# Autodesk Inventor assembly: E001-Chambre
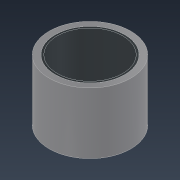
[picture p0: Inventor's stored thumbnail of the model, 180x180]
Saved by Autodesk Inventor 2021.3 (Build 253353000, 353)
## iProperties
Created: 2022-03-31
Part Number: E001-Chambre
Document SubType Name: Assembly
Designer: remi
Author: remi
## Documents named in this file (3)
- C:\Users\remi\OneDrive\Documents\Cours\05-HEVS\S2fb\mechanic\CCo\project\Compressor\E001-Chambre.iam
- C:\Users\remi\OneDrive\Documents\Cours\05-HEVS\S2fb\mechanic\CCo\project\Compressor\P002-Bati_chambre.ipt
- C:\Users\remi\OneDrive\Documents\Cours\05-HEVS\S2fb\mechanic\CCo\project\Compressor\P001-Couverture.ipt
## Components (2 placed, 2 different names)
1. P002-Bati_chambre:1 — Mate:1, Flush:1
2. P001-Couverture:1 — Mate:1, Flush:1
## Relationships (2: Mate 1, Flush 1)
- Mate:1: P002-Bati_chambre:1 ↔ P001-Couverture:1
- Flush:1: P002-Bati_chambre:1 ↔ P001-Couverture:1
